# Autodesk Inventor assembly: Ensamblaje1
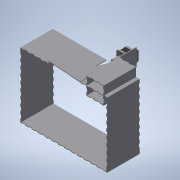
[picture p0: Inventor's stored thumbnail of the model, 180x180]
Saved by Autodesk Inventor 2020 (Build 240168000, 168)
## iProperties
Created: 2020-03-08
Part Number: Ensamblaje1
Material: Genérico
Document SubType Name: Assembly
Designer: Diego Guillén
Author: Diego Guillén
## Documents named in this file (11)
- C:\Users\joser\OneDrive\Documentos\UVG\2020\Digital 2\Proyecto\Maqueta\Guillen\Ensamblaje1.iam
- C:\Users\joser\OneDrive\Documentos\UVG\2020\Digital 2\Proyecto\Maqueta\Guillen\Pared1.ipt
- C:\Users\joser\OneDrive\Documentos\UVG\2020\Digital 2\Proyecto\Maqueta\Guillen\Pared2.ipt
- C:\Users\joser\OneDrive\Documentos\UVG\2020\Digital 2\Proyecto\Maqueta\Guillen\ParedFrontal.ipt
- C:\Users\joser\OneDrive\Documentos\UVG\2020\Digital 2\Proyecto\Maqueta\Guillen\stepper_bracket.ipt
- C:\Users\joser\OneDrive\Documentos\UVG\2020\Digital 2\Proyecto\Maqueta\Guillen\stepperStepper Motor 24VDC NEMA 17 42mm.ipt
- C:\Users\joser\OneDrive\Documentos\UVG\2020\Digital 2\Proyecto\Maqueta\Guillen\Pared Garita.ipt
- C:\Users\joser\OneDrive\Documentos\UVG\2020\Digital 2\Proyecto\Maqueta\Guillen\Pared Garita2.ipt
- C:\Users\joser\OneDrive\Documentos\UVG\2020\Digital 2\Proyecto\Maqueta\Guillen\Pared Garita3.ipt
- C:\Users\joser\OneDrive\Documentos\UVG\2020\Digital 2\Proyecto\Maqueta\Guillen\Porton.ipt
- C:\Users\joser\OneDrive\Documentos\UVG\2020\Digital 2\Proyecto\Maqueta\Guillen\Coupler 5x8.ipt
## Components (12 placed, 10 different names)
1. Pared1:1 — Coincidencia:2, Nivelación:1, Nivelación:2, Coincidencia:3, Nivelación:3, Nivelación:4
2. Pared2:1 — Coincidencia:2, Nivelación:1, Nivelación:2
3. Pared2:2 — Coincidencia:3, Nivelación:3, Nivelación:4, Nivelación:5, Nivelación:6, Nivelación:7
4. ParedFrontal:1 — Nivelación:5, Nivelación:6, Nivelación:7, Coincidencia:11, Coincidencia:12, Coincidencia:13, Nivelación:17, Coincidencia:19
5. stepper_bracket:1 — Coincidencia:4, Coincidencia:5, Coincidencia:6, Coincidencia:10, Nivelación:19
6. stepperStepper Motor 24VDC NEMA 17 42mm:1 — Coincidencia:4, Coincidencia:5, Coincidencia:6, Coincidencia:15, Coincidencia:16
7. Pared Garita:1 — Nivelación:12, Coincidencia:9, Nivelación:13
8. Pared Garita:2 — Coincidencia:7, Nivelación:8, Nivelación:9, Nivelación:10, Coincidencia:8, Nivelación:14
9. Pared Garita2:1 — Nivelación:10, Coincidencia:8, Nivelación:12, Coincidencia:9, Nivelación:13, Nivelación:14, Coincidencia:12
10. Pared Garita3:1 — Coincidencia:7, Nivelación:8, Nivelación:9, Coincidencia:10, Coincidencia:11, Coincidencia:13, Nivelación:19
11. Porton:1 — Nivelación:17, Coincidencia:17, Coincidencia:18
12. Coupler 5x8:1 — Coincidencia:15, Coincidencia:16, Coincidencia:17, Coincidencia:18, Coincidencia:19
## Relationships (32: Mate 17, Flush 15)
- Coincidencia:2 [Mate]: Pared1:1 ↔ Pared2:1
- Nivelación:1 [Flush]: Pared1:1 ↔ Pared2:1
- Nivelación:2 [Flush]: Pared1:1 ↔ Pared2:1
- Coincidencia:3 [Mate]: Pared1:1 ↔ Pared2:2
- Nivelación:3 [Flush]: Pared1:1 ↔ Pared2:2
- Nivelación:4 [Flush]: Pared1:1 ↔ Pared2:2
- Nivelación:5 [Flush]: Pared2:2 ↔ ParedFrontal:1
- Nivelación:6 [Flush]: Pared2:2 ↔ ParedFrontal:1
- Nivelación:7 [Flush]: Pared2:2 ↔ ParedFrontal:1
- Coincidencia:4 [Mate]: stepper_bracket:1 ↔ stepperStepper Motor 24VDC NEMA 17 42mm:1
- Coincidencia:5 [Mate]: stepper_bracket:1 ↔ stepperStepper Motor 24VDC NEMA 17 42mm:1
- Coincidencia:6 [Mate]: stepper_bracket:1 ↔ stepperStepper Motor 24VDC NEMA 17 42mm:1
- Coincidencia:7 [Mate]: Pared Garita:2 ↔ Pared Garita3:1
- Nivelación:8 [Flush]: Pared Garita:2 ↔ Pared Garita3:1
- Nivelación:9 [Flush]: Pared Garita:2 ↔ Pared Garita3:1
- Nivelación:10 [Flush]: Pared Garita:2 ↔ Pared Garita2:1
- Coincidencia:8 [Mate]: Pared Garita:2 ↔ Pared Garita2:1
- Nivelación:12 [Flush]: Pared Garita:1 ↔ Pared Garita2:1
- Coincidencia:9 [Mate]: Pared Garita:1 ↔ Pared Garita2:1
- Nivelación:13 [Flush]: Pared Garita:1 ↔ Pared Garita2:1
- Nivelación:14 [Flush]: Pared Garita:2 ↔ Pared Garita2:1
- Coincidencia:10 [Mate]: stepper_bracket:1 ↔ Pared Garita3:1
- Coincidencia:11 [Mate]: ParedFrontal:1 ↔ Pared Garita3:1
- Coincidencia:12 [Mate]: ParedFrontal:1 ↔ Pared Garita2:1
- Coincidencia:13 [Mate]: ParedFrontal:1 ↔ Pared Garita3:1
- Nivelación:17 [Flush]: ParedFrontal:1 ↔ Porton:1
- Coincidencia:15 [Mate]: stepperStepper Motor 24VDC NEMA 17 42mm:1 ↔ Coupler 5x8:1
- Nivelación:19 [Flush] (15 mm): stepper_bracket:1 ↔ Pared Garita3:1
- Coincidencia:16 [Mate]: stepperStepper Motor 24VDC NEMA 17 42mm:1 ↔ Coupler 5x8:1
- Coincidencia:17 [Mate]: Porton:1 ↔ Coupler 5x8:1
- Coincidencia:18 [Mate]: Porton:1 ↔ Coupler 5x8:1
- Coincidencia:19 [Mate] (5 mm): ParedFrontal:1 ↔ Coupler 5x8:1
